# Autodesk Inventor assembly: Assembly
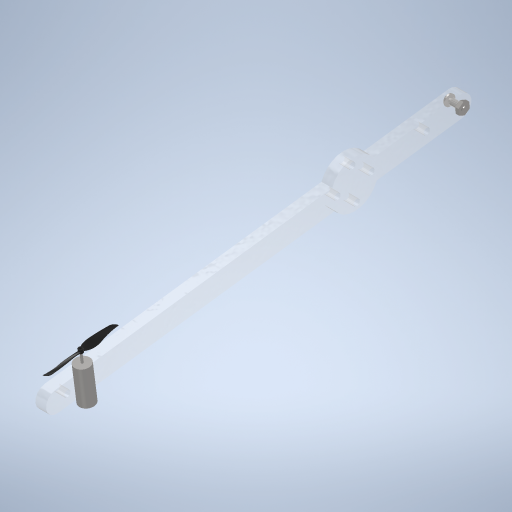
[picture p0: Inventor's stored thumbnail of the model, 512x512]
Saved by Autodesk Inventor 2023.1 (Build 271208000, 208)
## iProperties
Created: 2023-05-07
Part Number: Assembly
Document SubType Name: Assembly
Designer: felip
Author: felip
## Documents named in this file (6)
- C:\Users\felip\OneDrive\UNAL FORE\SEMESTRE 9\TECNICAS DE CONTROL\PROYECTO\PROYECTO-TDC-INVENTOR\Assembly - arm.iam
- C:\Users\felip\OneDrive\UNAL FORE\SEMESTRE 9\TECNICAS DE CONTROL\PROYECTO\PROYECTO-TDC-INVENTOR\brazo.ipt
- C:\Users\felip\OneDrive\UNAL FORE\SEMESTRE 9\TECNICAS DE CONTROL\PROYECTO\PROYECTO-TDC-INVENTOR\motor.ipt
- C:\Users\felip\OneDrive\UNAL FORE\SEMESTRE 9\TECNICAS DE CONTROL\PROYECTO\PROYECTO-TDC-INVENTOR\helice.ipt
- C:\Users\felip\OneDrive\Documents\Inventor\Content Center Files\R2023\en-US\BS 4183(4)\BS 4183 - M2,5 x 7(1) III.ipt
- C:\Users\felip\OneDrive\Documents\Inventor\Content Center Files\R2023\en-US\BS 4183(1)\BS 4183 - M2,5(1).ipt
## Components (5 placed, 5 different names)
1. brazo:1 — Flush:1, Tangent:1, Tangent:2, Insert:38, Insert:66
2. motor:1 — Flush:1, Tangent:1, Angle:1, Mate:7, Rotational:17
3. helice:1 — Rotational:17
4. BS 4183 Specification for machine screws and machine screw nuts. Metric series - Metric M2,5 x 7:1 — Insert:38
5. BS 4183 - Metric M2,5:7 — Insert:66
## Relationships (8: Tangent 2, Insert 2, Flush 1, Angle 1, Mate 1, RevoluteJoint 1)
- Flush:1: brazo:1 ↔ motor:1
- Tangent:1: brazo:1 ↔ motor:1
- Angle:1 (0 deg): motor:1
- Tangent:2: brazo:1
- Mate:7 (-15.5 mm): motor:1
- Rotational:17 [RevoluteJoint]: motor:1 ↔ helice:1
- Insert:38: brazo:1 ↔ BS 4183 Specification for machine screws and machine screw nuts. Metric series - Metric M2,5 x 7:1
- Insert:66: brazo:1 ↔ BS 4183 - Metric M2,5:7
